# Autodesk Inventor assembly: Microwave Detection Region
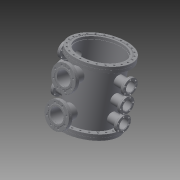
[picture p0: Inventor's stored thumbnail of the model, 180x180]
Saved by Autodesk Inventor 2015 (Build 190159000, 159)
## iProperties
Created: 2014-05-15
Part Number: Microwave Detection Region
Document SubType Name: Assembly
Designer: ijs09
Author: ijs09
## Documents named in this file (5)
- D:\Inventor\CCM CAD Files\CADFiles\EDM Machine\Microwave Detection Region\Microwave Detection Region.iam
- D:\Inventor\CCM CAD Files\CADFiles\EDM Machine\Microwave Detection Region\Detection Region Vacuum Collar.ipt
- D:\Inventor\CCM CAD Files\CADFiles\EDM Machine\Microwave Detection Region\DN200CF.ipt
- D:\Inventor\CCM CAD Files\CADFiles\EDM Machine\Microwave Detection Region\DN35CF Counter Bored.ipt
- D:\Inventor\CCM CAD Files\CADFiles\EDM Machine\Microwave Detection Region\DN63CF Counter Bored.ipt
## Components (11 placed, 4 different names)
1. Detection Region Vacuum Collar:1 — Mate:24, Mate:25, Mate:26, Mate:27, Mate:28, Mate:30, Mate:31, Mate:32, Mate:33, Mate:34, Mate:35, Mate:36, Mate:37, Mate:38, Mate:39, Mate:40, Mate:41, Mate:42, Mate:43, Mate:44
2. DN200CF:1 — Mate:24, Mate:25
3. DN200CF:2 — Mate:26, Mate:27
4. DN35CF Counter Bored:1 — Mate:28, Symmetry:1, Mate:31
5. DN35CF Counter Bored:2 — Mate:30, Symmetry:1, Mate:32
6. DN63CF Counter Bored:1 — Mate:35, Mate:36
7. DN63CF Counter Bored:2 — Mate:33, Mate:34
8. DN35CF Counter Bored:3 — Mate:37, Mate:38
9. DN35CF Counter Bored:4 — Mate:39, Mate:40
10. DN35CF Counter Bored:5 — Mate:41, Mate:42
11. DN35CF Counter Bored:6 — Mate:43, Mate:44
## Relationships (21: Mate 20, Symmetry 1)
- Mate:24: Detection Region Vacuum Collar:1 ↔ DN200CF:1
- Mate:25: Detection Region Vacuum Collar:1 ↔ DN200CF:1
- Mate:26: Detection Region Vacuum Collar:1 ↔ DN200CF:2
- Mate:27: Detection Region Vacuum Collar:1 ↔ DN200CF:2
- Mate:28: Detection Region Vacuum Collar:1 ↔ DN35CF Counter Bored:1
- Mate:30: Detection Region Vacuum Collar:1 ↔ DN35CF Counter Bored:2
- Symmetry:1: DN35CF Counter Bored:1 ↔ DN35CF Counter Bored:2
- Mate:31: Detection Region Vacuum Collar:1 ↔ DN35CF Counter Bored:1
- Mate:32: Detection Region Vacuum Collar:1 ↔ DN35CF Counter Bored:2
- Mate:33: Detection Region Vacuum Collar:1 ↔ DN63CF Counter Bored:2
- Mate:34: Detection Region Vacuum Collar:1 ↔ DN63CF Counter Bored:2
- Mate:35: Detection Region Vacuum Collar:1 ↔ DN63CF Counter Bored:1
- Mate:36: Detection Region Vacuum Collar:1 ↔ DN63CF Counter Bored:1
- Mate:37: Detection Region Vacuum Collar:1 ↔ DN35CF Counter Bored:3
- Mate:38: Detection Region Vacuum Collar:1 ↔ DN35CF Counter Bored:3
- Mate:39: Detection Region Vacuum Collar:1 ↔ DN35CF Counter Bored:4
- Mate:40: Detection Region Vacuum Collar:1 ↔ DN35CF Counter Bored:4
- Mate:41: Detection Region Vacuum Collar:1 ↔ DN35CF Counter Bored:5
- Mate:42: Detection Region Vacuum Collar:1 ↔ DN35CF Counter Bored:5
- Mate:43: Detection Region Vacuum Collar:1 ↔ DN35CF Counter Bored:6
- Mate:44: Detection Region Vacuum Collar:1 ↔ DN35CF Counter Bored:6
